# Autodesk Inventor assembly: LPTL_ASSEMBLY_2
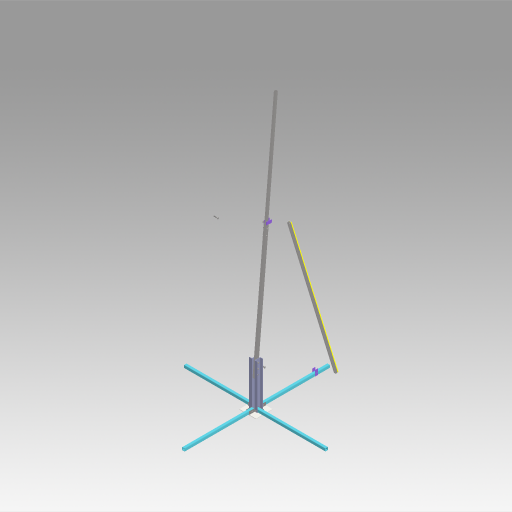
[picture p0: Inventor's stored thumbnail of the model, 512x512]
Saved by Autodesk Inventor 2023 (Build 270158000, 158)
## iProperties
Created: 2025-04-11
Part Number: LPTL_ASSEMBLY_2
Document SubType Name: Weldment
Designer: NELLY NDUNG'U
Mass: 80655.2 g
Surface Area: 40624.6 cm^2
Volume: 10274.5 cm^3
Density: 7.85 g/cm^3
Weld Material: Aluminum 6061, Welded
Author: NELLY NDUNG'U
## Documents named in this file (16)
- N:\NAKUJA\CAD FILES\AIRFRAME\LP003\LPTL_ASSEMBLY_2.iam
- N:\NAKUJA\CAD FILES\AIRFRAME\LP003\BASE_ASSEMBLY.iam
- N:\NAKUJA\CAD FILES\AIRFRAME\LP003\TL_50_40.iam
- C:\Users\User\Documents\Inventor\Content Center Files\R2023\en-US\ANSI B18.2.3.5M\ANSI B18.2.3.5M - M16 x 2 x 80.ipt
- C:\Users\User\Documents\Inventor\Content Center Files\R2023\en-US\ANSI B 18.2.4.1 M(1)\ANSI B 18.2.4.1 M - M16 x 2Style 1.ipt
- N:\NAKUJA\CAD FILES\AIRFRAME\LP003\SUPPORT ATTACHMENT.ipt
- N:\NAKUJA\CAD FILES\AIRFRAME\LP003\ENFORCEMENT.iam
- C:\Users\User\Documents\Inventor\Content Center Files\R2023\en-US\ANSI B18.2.3.5M\ANSI B18.2.3.5M - M16 x 2 x 65.ipt
- N:\NAKUJA\CAD FILES\AIRFRAME\LP003\LPTL_ASSEMBLY_2\AIP\FEA\f1ap77juo.fins
- N:\NAKUJA\CAD FILES\AIRFRAME\LP003\LPTL_ASSEMBLY_2\AIP\FEA\f1ap77jvk.fsat
- N:\NAKUJA\CAD FILES\AIRFRAME\LP003\LPTL_ASSEMBLY_2\AIP\FEA\f1ap77jvk.ftes
- N:\NAKUJA\CAD FILES\AIRFRAME\LP003\LPTL_ASSEMBLY_2\AIP\FEA\f1ap77jvk.fwiz
- N:\NAKUJA\CAD FILES\AIRFRAME\LP003\LPTL_ASSEMBLY_2\AIP\FEA\f1ap77khs.fmsh
- N:\NAKUJA\CAD FILES\AIRFRAME\LP003\LPTL_ASSEMBLY_2\AIP\FEA\f1ap77kio.fres
- N:\NAKUJA\CAD FILES\AIRFRAME\LP003\LPTL_ASSEMBLY_2\AIP\FEA\f1ap77lmo.fmsh
- N:\NAKUJA\CAD FILES\AIRFRAME\LP003\LPTL_ASSEMBLY_2\AIP\FEA\f1ap77lmp.fres
## Components (17 placed, 7 different names)
1. BASE_ASSEMBLY:1 [sub-assembly] — Angle:1, Mate:1, Mate:2, Mate:3, Insert:1, Insert:2, Insert:3, Insert:4, Insert:5, Insert:6, Flush:1, Mate:5, Mate:6, Mate:7, Flush:2, Mate:10, Mate:15, Mate:17
2. TL_50_40:1 [sub-assembly] — Angle:1, Mate:1, Mate:2, Mate:3, Flush:4, Mate:9, Flush:5, Mate:11
3. Hex Bolt - Metric M16 x 2 x 80:1 — Insert:1
4. Hex Bolt - Metric M16 x 2 x 80:2 — Insert:2
5. Hex Bolt - Metric M16 x 2 x 80:3 — Insert:3
6. Hex Nut Metric M16 x 2:1 — Insert:4
7. Hex Nut Metric M16 x 2:2 — Insert:5
8. Hex Nut Metric M16 x 2:3 — Insert:6
9. SUPPORT ATTACHMENT:1 — Mate:10, Flush:5, Mate:11
10. SUPPORT ATTACHMENT:2 — Flush:4, Mate:9, Mate:17
11. SUPPORT ATTACHMENT:3 — Mate:6, Mate:7, Flush:2
12. SUPPORT ATTACHMENT:4 — Flush:1, Mate:5, Mate:15
13. ENFORCEMENT:1 [sub-assembly]
14. Hex Bolt - Metric M16 x 2 x 65:2
15. Hex Bolt - Metric M16 x 2 x 65:1
16. Hex Nut Metric M16 x 2:4
17. Hex Nut Metric M16 x 2:5
## Relationships (22: Mate 11, Insert 6, Flush 4, Angle 1)
- Angle:1 (85 deg): BASE_ASSEMBLY:1 ↔ TL_50_40:1
- Mate:1 (-300 mm): BASE_ASSEMBLY:1 ↔ TL_50_40:1
- Mate:2: BASE_ASSEMBLY:1 ↔ TL_50_40:1
- Mate:3 (-8 mm): BASE_ASSEMBLY:1 ↔ TL_50_40:1
- Insert:1: BASE_ASSEMBLY:1 ↔ Hex Bolt - Metric M16 x 2 x 80:1
- Insert:2: BASE_ASSEMBLY:1 ↔ Hex Bolt - Metric M16 x 2 x 80:2
- Insert:3: BASE_ASSEMBLY:1 ↔ Hex Bolt - Metric M16 x 2 x 80:3
- Insert:4: BASE_ASSEMBLY:1 ↔ Hex Nut Metric M16 x 2:1
- Insert:5: BASE_ASSEMBLY:1 ↔ Hex Nut Metric M16 x 2:2
- Insert:6: BASE_ASSEMBLY:1 ↔ Hex Nut Metric M16 x 2:3
- Flush:1: BASE_ASSEMBLY:1 ↔ SUPPORT ATTACHMENT:4
- Mate:5 (990 mm): BASE_ASSEMBLY:1 ↔ SUPPORT ATTACHMENT:4
- Mate:6 (-5 mm): BASE_ASSEMBLY:1 ↔ SUPPORT ATTACHMENT:3
- Mate:7 (990 mm): BASE_ASSEMBLY:1 ↔ SUPPORT ATTACHMENT:3
- Flush:2: BASE_ASSEMBLY:1 ↔ SUPPORT ATTACHMENT:3
- Flush:4: TL_50_40:1 ↔ SUPPORT ATTACHMENT:2
- Mate:9: TL_50_40:1 ↔ SUPPORT ATTACHMENT:2
- Mate:10 (2750 mm): BASE_ASSEMBLY:1 ↔ SUPPORT ATTACHMENT:1
- Flush:5: TL_50_40:1 ↔ SUPPORT ATTACHMENT:1
- Mate:11: TL_50_40:1 ↔ SUPPORT ATTACHMENT:1
- Mate:15 (-5 mm): BASE_ASSEMBLY:1 ↔ SUPPORT ATTACHMENT:4
- Mate:17 (2750 mm): BASE_ASSEMBLY:1 ↔ SUPPORT ATTACHMENT:2
## Named parameters: sa_0 = 412500, sa_1 = 30000
note: some values were not read from the file. Shown as the stored number, unit unknown: "sa_0", "sa_1".
